# Autodesk Inventor assembly: Test_001
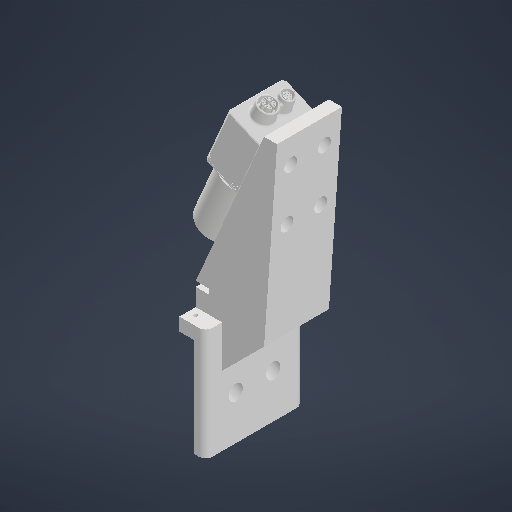
[picture p0: Inventor's stored thumbnail of the model, 512x512]
Saved by Autodesk Inventor 2026 (Build 300175000, 175)
## iProperties
Created: 2025-04-19
Part Number: Test_001
Document SubType Name: Assembly
Designer: Charl
Author: Charl
## Documents named in this file (3)
- E:\School\Research\Inventor\Cover\Test_001.iam
- E:\School\Research\Inventor\Cover\Camera_Bracket_Uru_001.ipt
- E:\School\Research\Inventor\Cover\Camera\Triton2_asm.iam
## Components (2 placed, 2 different names)
1. Camera_Bracket_Uru_001:1 — Mate:1, Mate:2
2. Triton2_asm:1 [sub-assembly] — Mate:1, Mate:2
## Relationships (2: Mate 2)
- Mate:1: Camera_Bracket_Uru_001:1 ↔ Triton2_asm:1
- Mate:2: Camera_Bracket_Uru_001:1 ↔ Triton2_asm:1
